# Autodesk Inventor assembly: Setup_1_part_2
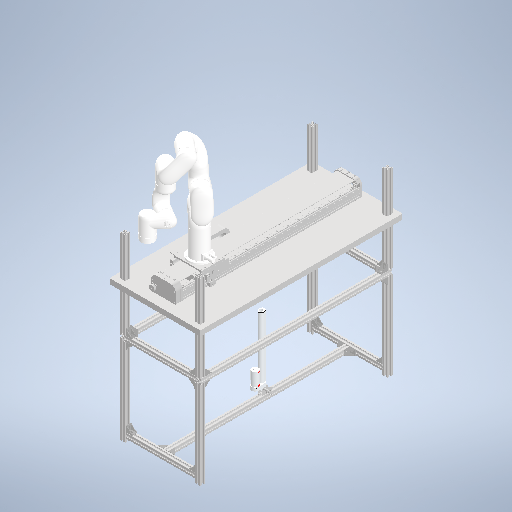
[picture p0: Inventor's stored thumbnail of the model, 512x512]
Saved by Autodesk Inventor 2025 (Build 290162000, 162)
## iProperties
Created: 2024-06-25
Part Number: Setup_1_part_2
Document SubType Name: Assembly
Designer: User
Author: User
## Documents named in this file (12)
- C:\Users\User\OneDrive\Documents\FYP\Inventor_Designs\Setup_1_part_2.iam
- C:\Users\User\OneDrive\Documents\FYP\Inventor_Designs\Metal Profile\Metal Profile 110 cm.ipt
- C:\Users\User\OneDrive\Documents\FYP\Inventor_Designs\Metal Profile\Metal Profile 40 cm.ipt
- C:\Users\User\OneDrive\Documents\FYP\Inventor_Designs\Metal Profile\Metal Profile 50 cm.ipt
- C:\Users\User\OneDrive\Documents\FYP\Inventor_Designs\Metal Profile\Metal Profile 104 cm.ipt
- C:\Users\User\OneDrive\Documents\FYP\Inventor_Designs\Triangle Bracket\Triangle Bracket.ipt
- C:\Users\User\OneDrive\Documents\FYP\Inventor_Designs\Linear Actuator\300mm Body.ipt
- C:\Users\User\OneDrive\Documents\FYP\Inventor_Designs\Clevis Pin\Celvis Pin.ipt
- C:\Users\User\OneDrive\Documents\FYP\Inventor_Designs\L Bracket\L Angle Bracket 30x30.ipt
- C:\Users\User\OneDrive\Documents\FYP\Inventor_Designs\Platform\Platform_Arm_2.ipt
- C:\Users\User\OneDrive\Documents\FYP\Inventor_Designs\Linear Motor\Motor.ipt
- C:\Users\User\OneDrive\Documents\FYP\Inventor_Designs\Designs_Arm\Arm.iam
## Components (49 placed, 11 different names)
1. Metal Profile 110 cm:1
2. Metal Profile 40 cm:1
3. Metal Profile 110 cm:2
4. Metal Profile 40 cm:2
5. Metal Profile 50 cm:1
6. Metal Profile 50 cm:2
7. Metal Profile 50 cm:3
8. Metal Profile 50 cm:4
9. Metal Profile 40 cm:3
10. Metal Profile 40 cm:4
11. Metal Profile 50 cm:5
12. Metal Profile 50 cm:6 — Mate:95, Mate:96
13. Metal Profile 50 cm:7
14. Metal Profile 50 cm:8
15. Metal Profile 104 cm:1
16. Triangle Bracket:1
17. 300mm Body:1
18. Celvis Pin:1
19. L Angle Bracket 30x30:1
20. L Angle Bracket 30x30:2
21. L Angle Bracket 30x30:3
22. L Angle Bracket 30x30:4
23. L Angle Bracket 30x30:5
24. L Angle Bracket 30x30:6
25. L Angle Bracket 30x30:7
26. L Angle Bracket 30x30:8
27. L Angle Bracket 30x30:9
28. L Angle Bracket 30x30:10
29. L Angle Bracket 30x30:11
30. L Angle Bracket 30x30:12
31. L Angle Bracket 30x30:13
32. L Angle Bracket 30x30:14
33. L Angle Bracket 30x30:15
34. L Angle Bracket 30x30:16
35. L Angle Bracket 30x30:17
36. L Angle Bracket 30x30:18
37. L Angle Bracket 30x30:19
38. L Angle Bracket 30x30:20
39. L Angle Bracket 30x30:21
40. L Angle Bracket 30x30:22
41. L Angle Bracket 30x30:23
42. L Angle Bracket 30x30:24
43. L Angle Bracket 30x30:25
44. L Angle Bracket 30x30:26
45. L Angle Bracket 30x30:27
46. L Angle Bracket 30x30:28
47. Platform_Arm_2:1 — Mate:95, Mate:96, Mate:100
48. Motor:1 — Mate:100
49. Arm:1 [sub-assembly]
## Relationships (109: Mate 100, Flush 8, Insert 1)
- [Mate]: Metal Profile 110 cm:1 ↔ Metal Profile 40 cm:1
- [Mate]: Metal Profile 40 cm:1 ↔ Metal Profile 110 cm:2
- [Mate]: Metal Profile 110 cm:1 ↔ Metal Profile 40 cm:1
- [Flush]: Metal Profile 110 cm:1 ↔ Metal Profile 40 cm:1
- [Flush]: Metal Profile 40 cm:1 ↔ Metal Profile 110 cm:2
- [Mate]: Metal Profile 110 cm:1 ↔ Metal Profile 40 cm:2
- [Flush]: Metal Profile 110 cm:1 ↔ Metal Profile 40 cm:1
- [Mate]: Metal Profile 110 cm:2 ↔ Metal Profile 40 cm:2
- [Flush]: Metal Profile 110 cm:2 ↔ Metal Profile 40 cm:2
- [Mate]: Metal Profile 110 cm:1 ↔ Metal Profile 40 cm:1
- [Mate]: Metal Profile 110 cm:1 ↔ Metal Profile 50 cm:1
- [Mate]: Metal Profile 110 cm:1 ↔ Metal Profile 50 cm:1
- [Flush]: Metal Profile 110 cm:1 ↔ Metal Profile 50 cm:1
- [Mate]: Metal Profile 110 cm:2 ↔ Metal Profile 50 cm:2
- [Mate]: Metal Profile 110 cm:2 ↔ Metal Profile 50 cm:2
- [Mate]: Metal Profile 110 cm:2 ↔ Metal Profile 50 cm:2
- [Mate]: Metal Profile 110 cm:2 ↔ Metal Profile 50 cm:4
- [Mate]: Metal Profile 110 cm:2 ↔ Metal Profile 50 cm:4
- [Mate]: Metal Profile 110 cm:2 ↔ Metal Profile 50 cm:4
- [Mate]: Metal Profile 110 cm:1 ↔ Metal Profile 50 cm:3
- [Mate]: Metal Profile 110 cm:1 ↔ Metal Profile 50 cm:3
- [Mate]: Metal Profile 110 cm:1 ↔ Metal Profile 50 cm:3
- [Mate]: Metal Profile 50 cm:3 ↔ Metal Profile 40 cm:3
- [Mate]: Metal Profile 50 cm:4 ↔ Metal Profile 40 cm:3
- [Mate] (450 mm): Metal Profile 40 cm:2 ↔ Metal Profile 40 cm:3
- [Mate]: Metal Profile 50 cm:2 ↔ Metal Profile 40 cm:4
- [Mate]: Metal Profile 50 cm:1 ↔ Metal Profile 40 cm:4
- [Mate] (450 mm): Metal Profile 40 cm:1 ↔ Metal Profile 40 cm:4
- [Mate]: Metal Profile 110 cm:2 ↔ Metal Profile 50 cm:6
- [Mate]: Metal Profile 50 cm:2 ↔ Metal Profile 50 cm:6
- [Mate]: Metal Profile 50 cm:2 ↔ Metal Profile 50 cm:6
- [Mate]: Metal Profile 50 cm:1 ↔ Metal Profile 50 cm:5
- [Mate]: Metal Profile 50 cm:1 ↔ Metal Profile 50 cm:5
- [Mate]: Metal Profile 50 cm:3 ↔ Metal Profile 50 cm:7
- [Mate]: Metal Profile 50 cm:3 ↔ Metal Profile 50 cm:7
- [Mate]: Metal Profile 50 cm:4 ↔ Metal Profile 50 cm:8
- [Mate]: Metal Profile 50 cm:4 ↔ Metal Profile 50 cm:8
- [Mate]: Metal Profile 110 cm:2 ↔ Metal Profile 50 cm:8
- [Mate]: Metal Profile 110 cm:1 ↔ Metal Profile 50 cm:7
- [Mate]: Metal Profile 110 cm:1 ↔ Metal Profile 50 cm:5
- [Mate] (185 mm): Metal Profile 40 cm:3 ↔ Metal Profile 104 cm:1
- [Mate]: Metal Profile 40 cm:3 ↔ Metal Profile 104 cm:1
- [Mate] (499 mm): Metal Profile 110 cm:2 ↔ Metal Profile 104 cm:1
- [Mate]: Metal Profile 104 cm:1 ↔ Triangle Bracket:1
- [Flush] (2 mm): Metal Profile 104 cm:1 ↔ Triangle Bracket:1
- [Flush] (570 mm): Metal Profile 40 cm:4 ↔ Triangle Bracket:1
- [Insert] (-22 mm): Triangle Bracket:1 ↔ 300mm Body:1
- [Mate]: Triangle Bracket:1 ↔ Celvis Pin:1
- [Mate]: Metal Profile 104 cm:1 ↔ L Angle Bracket 30x30:4
- [Mate]: Metal Profile 40 cm:4 ↔ L Angle Bracket 30x30:4
- [Mate]: Metal Profile 40 cm:3 ↔ L Angle Bracket 30x30:19
- [Mate]: Metal Profile 50 cm:3 ↔ L Angle Bracket 30x30:19
- [Mate]: Metal Profile 40 cm:4 ↔ L Angle Bracket 30x30:20
- [Mate]: Metal Profile 104 cm:1 ↔ L Angle Bracket 30x30:20
- [Mate]: Metal Profile 40 cm:3 ↔ L Angle Bracket 30x30:18
- [Mate]: Metal Profile 104 cm:1 ↔ L Angle Bracket 30x30:18
- [Mate]: Metal Profile 40 cm:3 ↔ L Angle Bracket 30x30:15
- [Mate]: Metal Profile 104 cm:1 ↔ L Angle Bracket 30x30:15
- [Mate]: Metal Profile 50 cm:1 ↔ L Angle Bracket 30x30:14
- [Mate]: Metal Profile 40 cm:4 ↔ L Angle Bracket 30x30:14
- [Mate]: Metal Profile 40 cm:4 ↔ L Angle Bracket 30x30:12
- [Mate]: Metal Profile 50 cm:2 ↔ L Angle Bracket 30x30:12
- [Mate]: Metal Profile 50 cm:2 ↔ L Angle Bracket 30x30:12
- [Mate]: Metal Profile 40 cm:3 ↔ L Angle Bracket 30x30:17
- [Mate]: Metal Profile 50 cm:4 ↔ L Angle Bracket 30x30:17
- [Mate]: Metal Profile 110 cm:1 ↔ L Angle Bracket 30x30:3
- [Mate]: Metal Profile 40 cm:1 ↔ L Angle Bracket 30x30:3
- [Mate]: Metal Profile 40 cm:1 ↔ L Angle Bracket 30x30:2
- [Mate]: Metal Profile 110 cm:2 ↔ L Angle Bracket 30x30:2
- [Mate]: Metal Profile 110 cm:1 ↔ L Angle Bracket 30x30:13
- [Mate]: Metal Profile 40 cm:2 ↔ L Angle Bracket 30x30:13
- [Mate]: Metal Profile 110 cm:2 ↔ L Angle Bracket 30x30:16
- [Mate]: Metal Profile 40 cm:2 ↔ L Angle Bracket 30x30:16
- [Mate]: Metal Profile 110 cm:2 ↔ L Angle Bracket 30x30:11
- [Mate]: Metal Profile 110 cm:2 ↔ L Angle Bracket 30x30:5
- [Flush]: Metal Profile 50 cm:2 ↔ L Angle Bracket 30x30:11
- [Mate]: Metal Profile 50 cm:4 ↔ L Angle Bracket 30x30:5
- [Mate]: Metal Profile 50 cm:3 ↔ L Angle Bracket 30x30:22
- [Mate]: Metal Profile 110 cm:1 ↔ L Angle Bracket 30x30:22
- [Mate]: Metal Profile 50 cm:1 ↔ L Angle Bracket 30x30:1
- [Mate]: Metal Profile 110 cm:1 ↔ L Angle Bracket 30x30:1
- [Mate]: Metal Profile 40 cm:1 ↔ L Angle Bracket 30x30:10
- [Mate]: Metal Profile 50 cm:2 ↔ L Angle Bracket 30x30:8
- [Mate]: Metal Profile 40 cm:1 ↔ L Angle Bracket 30x30:8
- [Mate]: Metal Profile 40 cm:2 ↔ L Angle Bracket 30x30:9
- [Mate]: Metal Profile 50 cm:4 ↔ L Angle Bracket 30x30:7
- [Mate]: Metal Profile 40 cm:2 ↔ L Angle Bracket 30x30:7
- [Mate]: Metal Profile 50 cm:8 ↔ L Angle Bracket 30x30:23
- [Mate]: Metal Profile 50 cm:8 ↔ L Angle Bracket 30x30:6
- [Mate]: Metal Profile 110 cm:2 ↔ L Angle Bracket 30x30:23
- [Mate]: Metal Profile 40 cm:2 ↔ L Angle Bracket 30x30:6
- [Mate]: Metal Profile 50 cm:7 ↔ L Angle Bracket 30x30:21
- [Mate]: Metal Profile 40 cm:2 ↔ L Angle Bracket 30x30:21
- [Mate]: Metal Profile 50 cm:7 ↔ L Angle Bracket 30x30:27
- [Mate]: Metal Profile 110 cm:1 ↔ L Angle Bracket 30x30:27
- [Mate]: Metal Profile 50 cm:6 ↔ L Angle Bracket 30x30:24
- [Mate]: Metal Profile 40 cm:1 ↔ L Angle Bracket 30x30:24
- [Mate]: Metal Profile 50 cm:5 ↔ L Angle Bracket 30x30:25
- [Mate]: Metal Profile 40 cm:1 ↔ L Angle Bracket 30x30:25
- [Mate]: Metal Profile 110 cm:1 ↔ L Angle Bracket 30x30:28
- [Mate]: Metal Profile 110 cm:2 ↔ L Angle Bracket 30x30:26
- [Mate]: Metal Profile 50 cm:6 ↔ L Angle Bracket 30x30:26
- [Mate]: Metal Profile 50 cm:5 ↔ L Angle Bracket 30x30:28
- Mate:95: Metal Profile 50 cm:6 ↔ Platform_Arm_2:1
- Mate:96: Metal Profile 50 cm:6 ↔ Platform_Arm_2:1
- [Mate]: Motor:1 ↔ Arm:1
- [Mate]: Motor:1 ↔ Arm:1
- [Mate]: Motor:1 ↔ Arm:1
- Mate:100: Platform_Arm_2:1 ↔ Motor:1
## Named parameters: d55_d86 = 0 mm, d56_d88 = 499 mm, d57_d101 = 0 mm, d58_d102 = 2 mm, d78_d85 = 185 mm
